# Autodesk Inventor assembly: BoronProbe_5
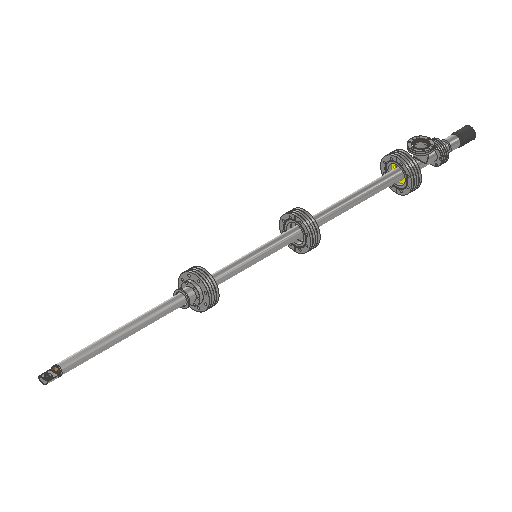
[picture p0: Inventor's stored thumbnail of the model, 512x512]
Saved by Autodesk Inventor 2026.2 (Build 302298000, 298)
## iProperties
Created: 2026-05-08
Part Number: BoronProbe_5
Document SubType Name: Assembly
Designer: zetsu
ProbePos: 738.000 mm
Author: zetsu
## Documents named in this file (26)
- D:\repos\PIHTI\BoronProbe_2026\BoronProbe_2026.iam
- D:\repos\PIHTI\BoronProbe_2026\parts\B_probehead_5.ipt
- D:\repos\PIHTI\BoronProbe_2026\parts\B_holder_sub_5.ipt
- D:\repos\PIHTI\BoronProbe_2026\parts\B_pipe_cylinder_5.ipt
- D:\repos\PIHTI\BoronProbe_2026\parts\M3x6-BHCS.ipt
- D:\repos\PIHTI\BoronProbe_2026\parts\ceramic_bushing_M3-v1.ipt
- D:\repos\PIHTI\BoronProbe_2026\parts\ceramic_washer_M4_v1.ipt
- D:\repos\PIHTI\BoronProbe_2026\parts\B_shield_5.iam
- D:\repos\PIHTI\BoronProbe_2026\parts\ceramic_spacer_d3-13.ipt
- D:\repos\PIHTI\BoronProbe_2026\parts\ceramic_2-hole-spacer_d3-13.ipt
- D:\repos\PIHTI\BoronProbe_2026\parts\M2-4_screw.ipt
- D:\repos\PIHTI\BoronProbe_2026\parts\ICF70TE\ICF70TE.iam
- D:\repos\PIHTI\BoronProbe_2026\parts\C25K22A4CU.iam
- D:\repos\PIHTI\BoronProbe_2026\parts\substrate.ipt
- D:\repos\PIHTI\BoronProbe_2026\parts\M3-nut.ipt
- D:\repos\PIHTI\BoronProbe_2026\parts\B_holder_up_5.ipt
- D:\repos\PIHTI\BoronProbe_2026\parts\B_probe_pipe_5.ipt
- D:\repos\PIHTI\BoronProbe_2026\parts\Rotary_Feedthrough\Rotary_Feedthrough.iam
- D:\repos\PIHTI\BoronProbe_2026\parts\M3x10-BHCS.ipt
- D:\repos\PIHTI\BoronProbe_2026\parts\M3x20-BHCS.ipt
- D:\repos\PIHTI\BoronProbe_2026\parts\ICF114-through.ipt
- D:\repos\PIHTI\BoronProbe_2026\parts\ICF70_to_KF40.ipt
- D:\repos\PIHTI\BoronProbe_2026\parts\B_probe_bearing.ipt
- D:\repos\PIHTI\BoronProbe_2026\parts\rotary_transfer_shaft_5_1.ipt
- D:\repos\PIHTI\BoronProbe_2026\parts\ICF_114-70_bearing.ipt
- D:\repos\PIHTI\BoronProbe_2026\parts\M4×12-VentedHexBolt.ipt
## Components (54 placed, 23 different names)
1. B_probehead_5:1 — メイト:1, メイト:2, メイト:3, メイト:4, メイト:6, メイト:12, メイト:13, メイト:14, メイト:15, メイト:16, メイト:17, メイト:18, メイト:20, メイト:22, メイト:49, メイト:50, メイト:51, メイト:53, フラッシュ:2, メイト:54, フラッシュ:3, メイト:55, フラッシュ:4
2. B_holder_sub_5:1 — メイト:1, メイト:2, メイト:3, メイト:5, メイト:7, メイト:76, メイト:77, メイト:78, メイト:79, メイト:80, メイト:81, メイト:82, メイト:83, メイト:86
3. Broached Hexagon Socket Button Head Cap Screw - Metric M3 x 0.5 x 6:1 — メイト:4, メイト:5
4. Broached Hexagon Socket Button Head Cap Screw - Metric M3 x 0.5 x 6:2 — メイト:6, メイト:7
5. Broached Hexagon Socket Button Head Cap Screw - Metric M3 x 0.5 x 6:5 — メイト:40, メイト:41
6. ceramic_bushing_M3-v1:1 — メイト:16, メイト:17, メイト:23, メイト:36, メイト:37
7. ceramic_bushing_M3-v1:2 — メイト:14, メイト:15, メイト:19, メイト:40, メイト:41
8. ceramic_bushing_M3-v1:3 — メイト:12, メイト:13, メイト:21, メイト:38, メイト:39
9. ceramic_washer_M4_v1:1 — メイト:20, メイト:21, メイト:43
10. ceramic_washer_M4_v1:2 — メイト:18, メイト:19, メイト:42
11. ceramic_washer_M4_v1:3 — メイト:22, メイト:23, メイト:44
12. Broached Hexagon Socket Button Head Cap Screw - Metric M3 x 0.5 x 6:6 — メイト:38, メイト:39
13. Broached Hexagon Socket Button Head Cap Screw - Metric M3 x 0.5 x 6:7 — メイト:36, メイト:37
14. B_pipe_cylinder_5:1 — メイト:42, メイト:43, メイト:44, メイト:93, メイト:94
15. B_shield_5:1 [sub-assembly] — メイト:49, メイト:50, メイト:51, メイト:56, メイト:57, メイト:58, メイト:59
16. ceramic_spacer_d3-13:1 — メイト:53, フラッシュ:2
17. ceramic_spacer_d3-13:2 — メイト:54, フラッシュ:3
18. ceramic_2-hole-spacer_d3-13:1 — メイト:55, フラッシュ:4
19. M2-4_screw:1 — メイト:56, メイト:57
20. M2-4_screw:2 — メイト:58, メイト:59
21. C25K22A4CU:1 [sub-assembly]
22. substrate:1 — メイト:76, メイト:77, メイト:84
23. JIS B 1181 Style 1 - Metric A M3:1 — メイト:78, メイト:79
24. JIS B 1181 Style 1 - Metric A M3:2 — メイト:82, メイト:83
25. JIS B 1181 Style 1 - Metric A M3:3 — メイト:80, メイト:81, メイト:85
26. B_holder_up_5:1 — メイト:84, メイト:85, メイト:86, メイト:87, メイト:88, メイト:89, メイト:90, メイト:91, メイト:92
27. Broached Hexagon Socket Button Head Cap Screw - Metric M3 x 0.5 x 6:8 — メイト:87, メイト:88
28. Broached Hexagon Socket Button Head Cap Screw - Metric M3 x 0.5 x 6:9 — メイト:89, メイト:90
29. Broached Hexagon Socket Button Head Cap Screw - Metric M3 x 0.5 x 6:10 — メイト:91, メイト:92
30. B_probe_pipe_5:1 — メイト:93, メイト:94, メイト:95, メイト:96, メイト:99, メイト:100, メイト:101, メイト:102, メイト:103, メイト:104, メイト:105, メイト:106
31. rotary_transfer_shaft_5_1:1 — メイト:95, メイト:96, メイト:97, メイト:98, メイト:116, メイト:117, メイト:119, メイト:142, メイト:143
32. Rotary_Feedthrough:1 [sub-assembly] — メイト:97, メイト:98, メイト:110, メイト:140, メイト:141
33. Broached Hexagon Socket Button Head Cap Screw - Metric M3 x 0.5 x 6:11 — メイト:99, メイト:100, メイト:142
34. Broached Hexagon Socket Button Head Cap Screw - Metric M3 x 0.5 x 6:12 — メイト:101, メイト:102, メイト:143
35. Broached Hexagon Socket Button Head Cap Screw - Metric M3 x 0.5 x 6:13 — メイト:103, メイト:104
36. Broached Hexagon Socket Button Head Cap Screw - Metric M3 x 0.5 x 6:14 — メイト:105, メイト:106
37. ICF70TE:2 [sub-assembly] — メイト:110, メイト:113, メイト:114, メイト:115, メイト:140, メイト:141
38. ICF_114-70_bearing:1 — メイト:113, メイト:114, メイト:115, メイト:121, メイト:122, メイト:135, メイト:136, メイト:137, メイト:144
39. Broached Hexagon Socket Button Head Cap Screw - Metric M3 x 0.5 x 6:15 — メイト:116, メイト:117, メイト:118
40. JIS B 1181 Style 1 - Metric A M3:4 — メイト:118, メイト:119
41. ICF114-through:1 — メイト:121, メイト:122, メイト:123, メイト:124, メイト:137, フラッシュ:5, フラッシュ:6
42. ICF114-through:2 — メイト:123, メイト:124, メイト:125, メイト:126, メイト:127, メイト:129
43. ICF114-through:3 — メイト:125, メイト:126, メイト:127, メイト:128, フラッシュ:5
44. ICF114-through:4 — メイト:128, メイト:129, メイト:130, メイト:131, メイト:132, 角度:1
45. ICF_114-70_bearing:2 — メイト:130, メイト:131, メイト:132, メイト:133, メイト:134, メイト:138, メイト:139, フラッシュ:6, メイト:151
46. ICF70_to_KF40:1 — メイト:133, メイト:134, 角度:1
47. B_probe_bearing:1 — メイト:135, メイト:136, メイト:144, メイト:145, メイト:146, メイト:147, メイト:148, メイト:149, メイト:150
48. B_probe_bearing:2 — メイト:138, メイト:139, メイト:151, メイト:152, メイト:153, メイト:154, メイト:155, メイト:156, メイト:157
49. M4×12-VentedHexBolt:1 — メイト:145, メイト:146
50. M4×12-VentedHexBolt:2 — メイト:147, メイト:148
51. M4×12-VentedHexBolt:3 — メイト:149, メイト:150
52. M4×12-VentedHexBolt:4 — メイト:152, メイト:153
53. M4×12-VentedHexBolt:5 — メイト:154, メイト:155
54. M4×12-VentedHexBolt:6 — メイト:156, メイト:157
## Relationships (120: Mate 114, Flush 5, Angle 1)
- メイト:1 [Mate]: B_probehead_5:1 ↔ B_holder_sub_5:1
- メイト:2 [Mate]: B_probehead_5:1 ↔ B_holder_sub_5:1
- メイト:3 [Mate]: B_probehead_5:1 ↔ B_holder_sub_5:1
- メイト:4 [Mate]: B_probehead_5:1 ↔ Broached Hexagon Socket Button Head Cap Screw - Metric M3 x 0.5 x 6:1
- メイト:5 [Mate]: B_holder_sub_5:1 ↔ Broached Hexagon Socket Button Head Cap Screw - Metric M3 x 0.5 x 6:1
- メイト:6 [Mate]: B_probehead_5:1 ↔ Broached Hexagon Socket Button Head Cap Screw - Metric M3 x 0.5 x 6:2
- メイト:7 [Mate]: B_holder_sub_5:1 ↔ Broached Hexagon Socket Button Head Cap Screw - Metric M3 x 0.5 x 6:2
- メイト:12 [Mate]: B_probehead_5:1 ↔ ceramic_bushing_M3-v1:3
- メイト:13 [Mate]: B_probehead_5:1 ↔ ceramic_bushing_M3-v1:3
- メイト:14 [Mate]: B_probehead_5:1 ↔ ceramic_bushing_M3-v1:2
- メイト:15 [Mate]: B_probehead_5:1 ↔ ceramic_bushing_M3-v1:2
- メイト:16 [Mate]: B_probehead_5:1 ↔ ceramic_bushing_M3-v1:1
- メイト:17 [Mate]: B_probehead_5:1 ↔ ceramic_bushing_M3-v1:1
- メイト:18 [Mate]: B_probehead_5:1 ↔ ceramic_washer_M4_v1:2
- メイト:19 [Mate]: ceramic_bushing_M3-v1:2 ↔ ceramic_washer_M4_v1:2
- メイト:20 [Mate]: B_probehead_5:1 ↔ ceramic_washer_M4_v1:1
- メイト:21 [Mate]: ceramic_bushing_M3-v1:3 ↔ ceramic_washer_M4_v1:1
- メイト:22 [Mate]: B_probehead_5:1 ↔ ceramic_washer_M4_v1:3
- メイト:23 [Mate]: ceramic_bushing_M3-v1:1 ↔ ceramic_washer_M4_v1:3
- メイト:36 [Mate]: ceramic_bushing_M3-v1:1 ↔ Broached Hexagon Socket Button Head Cap Screw - Metric M3 x 0.5 x 6:7
- メイト:37 [Mate]: ceramic_bushing_M3-v1:1 ↔ Broached Hexagon Socket Button Head Cap Screw - Metric M3 x 0.5 x 6:7
- メイト:38 [Mate]: ceramic_bushing_M3-v1:3 ↔ Broached Hexagon Socket Button Head Cap Screw - Metric M3 x 0.5 x 6:6
- メイト:39 [Mate]: ceramic_bushing_M3-v1:3 ↔ Broached Hexagon Socket Button Head Cap Screw - Metric M3 x 0.5 x 6:6
- メイト:40 [Mate]: Broached Hexagon Socket Button Head Cap Screw - Metric M3 x 0.5 x 6:5 ↔ ceramic_bushing_M3-v1:2
- メイト:41 [Mate]: Broached Hexagon Socket Button Head Cap Screw - Metric M3 x 0.5 x 6:5 ↔ ceramic_bushing_M3-v1:2
- メイト:42 [Mate]: ceramic_washer_M4_v1:2 ↔ B_pipe_cylinder_5:1
- メイト:43 [Mate]: ceramic_washer_M4_v1:1 ↔ B_pipe_cylinder_5:1
- メイト:44 [Mate]: ceramic_washer_M4_v1:3 ↔ B_pipe_cylinder_5:1
- メイト:49 [Mate]: B_probehead_5:1 ↔ B_shield_5:1
- メイト:50 [Mate]: B_probehead_5:1 ↔ B_shield_5:1
- メイト:51 [Mate]: B_probehead_5:1 ↔ B_shield_5:1
- メイト:53 [Mate]: B_probehead_5:1 ↔ ceramic_spacer_d3-13:1
- フラッシュ:2 [Flush]: B_probehead_5:1 ↔ ceramic_spacer_d3-13:1
- メイト:54 [Mate]: B_probehead_5:1 ↔ ceramic_spacer_d3-13:2
- フラッシュ:3 [Flush]: B_probehead_5:1 ↔ ceramic_spacer_d3-13:2
- メイト:55 [Mate]: B_probehead_5:1 ↔ ceramic_2-hole-spacer_d3-13:1
- フラッシュ:4 [Flush]: B_probehead_5:1 ↔ ceramic_2-hole-spacer_d3-13:1
- メイト:56 [Mate]: B_shield_5:1 ↔ M2-4_screw:1
- メイト:57 [Mate]: B_shield_5:1 ↔ M2-4_screw:1
- メイト:58 [Mate]: B_shield_5:1 ↔ M2-4_screw:2
- メイト:59 [Mate]: B_shield_5:1 ↔ M2-4_screw:2
- メイト:76 [Mate]: B_holder_sub_5:1 ↔ substrate:1
- メイト:77 [Mate]: B_holder_sub_5:1 ↔ substrate:1
- メイト:78 [Mate]: B_holder_sub_5:1 ↔ JIS B 1181 Style 1 - Metric A M3:1
- メイト:79 [Mate]: B_holder_sub_5:1 ↔ JIS B 1181 Style 1 - Metric A M3:1
- メイト:80 [Mate]: B_holder_sub_5:1 ↔ JIS B 1181 Style 1 - Metric A M3:3
- メイト:81 [Mate]: B_holder_sub_5:1 ↔ JIS B 1181 Style 1 - Metric A M3:3
- メイト:82 [Mate]: B_holder_sub_5:1 ↔ JIS B 1181 Style 1 - Metric A M3:2
- メイト:83 [Mate]: B_holder_sub_5:1 ↔ JIS B 1181 Style 1 - Metric A M3:2
- メイト:84 [Mate]: substrate:1 ↔ B_holder_up_5:1
- メイト:85 [Mate]: JIS B 1181 Style 1 - Metric A M3:3 ↔ B_holder_up_5:1
- メイト:86 [Mate]: B_holder_sub_5:1 ↔ B_holder_up_5:1
- メイト:87 [Mate]: B_holder_up_5:1 ↔ Broached Hexagon Socket Button Head Cap Screw - Metric M3 x 0.5 x 6:8
- メイト:88 [Mate]: B_holder_up_5:1 ↔ Broached Hexagon Socket Button Head Cap Screw - Metric M3 x 0.5 x 6:8
- メイト:89 [Mate]: B_holder_up_5:1 ↔ Broached Hexagon Socket Button Head Cap Screw - Metric M3 x 0.5 x 6:9
- メイト:90 [Mate]: B_holder_up_5:1 ↔ Broached Hexagon Socket Button Head Cap Screw - Metric M3 x 0.5 x 6:9
- メイト:91 [Mate]: B_holder_up_5:1 ↔ Broached Hexagon Socket Button Head Cap Screw - Metric M3 x 0.5 x 6:10
- メイト:92 [Mate]: B_holder_up_5:1 ↔ Broached Hexagon Socket Button Head Cap Screw - Metric M3 x 0.5 x 6:10
- メイト:93 [Mate]: B_pipe_cylinder_5:1 ↔ B_probe_pipe_5:1
- メイト:94 [Mate]: B_pipe_cylinder_5:1 ↔ B_probe_pipe_5:1
- メイト:95 [Mate]: B_probe_pipe_5:1 ↔ rotary_transfer_shaft_5_1:1
- メイト:96 [Mate]: B_probe_pipe_5:1 ↔ rotary_transfer_shaft_5_1:1
- メイト:97 [Mate]: rotary_transfer_shaft_5_1:1 ↔ Rotary_Feedthrough:1
- メイト:98 [Mate]: rotary_transfer_shaft_5_1:1 ↔ Rotary_Feedthrough:1
- メイト:99 [Mate]: B_probe_pipe_5:1 ↔ Broached Hexagon Socket Button Head Cap Screw - Metric M3 x 0.5 x 6:11
- メイト:100 [Mate]: B_probe_pipe_5:1 ↔ Broached Hexagon Socket Button Head Cap Screw - Metric M3 x 0.5 x 6:11
- メイト:101 [Mate]: B_probe_pipe_5:1 ↔ Broached Hexagon Socket Button Head Cap Screw - Metric M3 x 0.5 x 6:12
- メイト:102 [Mate]: B_probe_pipe_5:1 ↔ Broached Hexagon Socket Button Head Cap Screw - Metric M3 x 0.5 x 6:12
- メイト:103 [Mate]: B_probe_pipe_5:1 ↔ Broached Hexagon Socket Button Head Cap Screw - Metric M3 x 0.5 x 6:13
- メイト:104 [Mate]: B_probe_pipe_5:1 ↔ Broached Hexagon Socket Button Head Cap Screw - Metric M3 x 0.5 x 6:13
- メイト:105 [Mate]: B_probe_pipe_5:1 ↔ Broached Hexagon Socket Button Head Cap Screw - Metric M3 x 0.5 x 6:14
- メイト:106 [Mate]: B_probe_pipe_5:1 ↔ Broached Hexagon Socket Button Head Cap Screw - Metric M3 x 0.5 x 6:14
- メイト:110 [Mate]: Rotary_Feedthrough:1 ↔ ICF70TE:2
- メイト:113 [Mate]: ICF70TE:2 ↔ ICF_114-70_bearing:1
- メイト:114 [Mate]: ICF70TE:2 ↔ ICF_114-70_bearing:1
- メイト:115 [Mate]: ICF70TE:2 ↔ ICF_114-70_bearing:1
- メイト:116 [Mate]: rotary_transfer_shaft_5_1:1 ↔ Broached Hexagon Socket Button Head Cap Screw - Metric M3 x 0.5 x 6:15
- メイト:117 [Mate]: rotary_transfer_shaft_5_1:1 ↔ Broached Hexagon Socket Button Head Cap Screw - Metric M3 x 0.5 x 6:15
- メイト:118 [Mate]: Broached Hexagon Socket Button Head Cap Screw - Metric M3 x 0.5 x 6:15 ↔ JIS B 1181 Style 1 - Metric A M3:4
- メイト:119 [Mate]: rotary_transfer_shaft_5_1:1 ↔ JIS B 1181 Style 1 - Metric A M3:4
- メイト:121 [Mate]: ICF_114-70_bearing:1 ↔ ICF114-through:1
- メイト:122 [Mate]: ICF_114-70_bearing:1 ↔ ICF114-through:1
- メイト:123 [Mate]: ICF114-through:1 ↔ ICF114-through:2
- メイト:124 [Mate]: ICF114-through:1 ↔ ICF114-through:2
- メイト:125 [Mate]: ICF114-through:2 ↔ ICF114-through:3
- メイト:126 [Mate]: ICF114-through:2 ↔ ICF114-through:3
- メイト:127 [Mate]: ICF114-through:2 ↔ ICF114-through:3
- メイト:128 [Mate]: ICF114-through:3 ↔ ICF114-through:4
- メイト:129 [Mate]: ICF114-through:2 ↔ ICF114-through:4
- メイト:130 [Mate]: ICF114-through:4 ↔ ICF_114-70_bearing:2
- メイト:131 [Mate]: ICF114-through:4 ↔ ICF_114-70_bearing:2
- メイト:132 [Mate]: ICF114-through:4 ↔ ICF_114-70_bearing:2
- メイト:133 [Mate]: ICF_114-70_bearing:2 ↔ ICF70_to_KF40:1
- メイト:134 [Mate]: ICF_114-70_bearing:2 ↔ ICF70_to_KF40:1
- 角度:1 [Angle] (0 deg): ICF114-through:4 ↔ ICF70_to_KF40:1
- メイト:135 [Mate]: ICF_114-70_bearing:1 ↔ B_probe_bearing:1
- メイト:136 [Mate]: ICF_114-70_bearing:1 ↔ B_probe_bearing:1
- メイト:137 [Mate]: ICF_114-70_bearing:1 ↔ ICF114-through:1
- メイト:138 [Mate]: ICF_114-70_bearing:2 ↔ B_probe_bearing:2
- メイト:139 [Mate]: ICF_114-70_bearing:2 ↔ B_probe_bearing:2
- メイト:140 [Mate]: Rotary_Feedthrough:1 ↔ ICF70TE:2
- メイト:141 [Mate]: Rotary_Feedthrough:1 ↔ ICF70TE:2
- フラッシュ:5 [Flush] (369 mm): ICF114-through:1 ↔ ICF114-through:3
- メイト:142 [Mate]: rotary_transfer_shaft_5_1:1 ↔ Broached Hexagon Socket Button Head Cap Screw - Metric M3 x 0.5 x 6:11
- メイト:143 [Mate]: rotary_transfer_shaft_5_1:1 ↔ Broached Hexagon Socket Button Head Cap Screw - Metric M3 x 0.5 x 6:12
- フラッシュ:6 [Flush] (738 mm): ICF114-through:1 ↔ ICF_114-70_bearing:2
- メイト:144 [Mate]: ICF_114-70_bearing:1 ↔ B_probe_bearing:1
- メイト:145 [Mate]: B_probe_bearing:1 ↔ M4×12-VentedHexBolt:1
- メイト:146 [Mate]: B_probe_bearing:1 ↔ M4×12-VentedHexBolt:1
- メイト:147 [Mate]: B_probe_bearing:1 ↔ M4×12-VentedHexBolt:2
- メイト:148 [Mate]: B_probe_bearing:1 ↔ M4×12-VentedHexBolt:2
- メイト:149 [Mate]: B_probe_bearing:1 ↔ M4×12-VentedHexBolt:3
- メイト:150 [Mate]: B_probe_bearing:1 ↔ M4×12-VentedHexBolt:3
- メイト:151 [Mate]: ICF_114-70_bearing:2 ↔ B_probe_bearing:2
- メイト:152 [Mate]: B_probe_bearing:2 ↔ M4×12-VentedHexBolt:4
- メイト:153 [Mate]: B_probe_bearing:2 ↔ M4×12-VentedHexBolt:4
- メイト:154 [Mate]: B_probe_bearing:2 ↔ M4×12-VentedHexBolt:5
- メイト:155 [Mate]: B_probe_bearing:2 ↔ M4×12-VentedHexBolt:5
- メイト:156 [Mate]: B_probe_bearing:2 ↔ M4×12-VentedHexBolt:6
- メイト:157 [Mate]: B_probe_bearing:2 ↔ M4×12-VentedHexBolt:6
## Named parameters: ProbePos = 738 mm, ProbePos_Max = 410 mm, ProbePos_Min = 738 mm
